# Autodesk Inventor assembly: Vex Traction Wheel 4x2
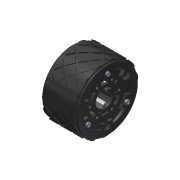
[picture p0: Inventor's stored thumbnail of the model, 180x180]
Saved by Autodesk Inventor 2013 (Build 170138000, 138)
## iProperties
Created: 2012-12-09
Part Number: Vex Traction Wheel 4x2
Document SubType Name: Assembly
Designer: Nemo
Author: Nemo
## Documents named in this file (7)
- H:\Nemo\Documents\Robotics\VexPro\Wheels\Assemblies\Vex Traction Wheel 4x2.iam
- H:\Nemo\Documents\Robotics\VexPro\Wheels\Components\Traction Tire Body 4in.ipt
- H:\Nemo\Documents\Robotics\VexPro\Wheels\Components\Traction Tire extension 4in.ipt
- H:\Nemo\Documents\Robotics\VexPro\Fasteners\8-32 locknut.ipt
- H:\Nemo\Documents\Robotics\VexPro\Fasteners\Hex Standoff 8-32 x1750.ipt
- H:\Nemo\Documents\Robotics\VexPro\Fasteners\8-32 SHCS x2250.ipt
- H:\Nemo\Documents\Robotics\VexPro\Wheels\Components\4 Traction Tire - 2 Wide.ipt
## Components (17 placed, 6 different names)
1. Traction Tire Body 4in:1 — Mate:1, Mate:2, Mate:3, Mate:4, Mate:5, Mate:6, Mate:9, Angle:1, Mate:10, Insert:2, Angle:2
2. Traction Tire Body 4in:2 — Mate:3, Mate:7, Insert:1, Mate:12, Insert:4
3. Traction Tire extension 4in:1 — Mate:4, Mate:5, Mate:6, Mate:7, Flush:1, Insert:3
4. Traction Tire extension 4in:2 — Mate:11, Insert:3, Mate:12
5. 4 Traction Tire - 2 Wide:1 — Mate:13, Mate:14, Mate:15
6. Hex Standoff 8-32 x1750:1 — Mate:9, Angle:1, Mate:10
7. Hex Standoff 8-32 x1750:2
8. Hex Standoff 8-32 x1750:3
9. Hex Standoff 8-32 x1750:4
10. Hex Standoff 8-32 x1750:5
11. Hex Standoff 8-32 x1750:6
12. 8-32 SHCS x2250:1 — Insert:1, Insert:4
13. 8-32 locknut:1 — Insert:2, Angle:2
14. 8-32 SHCS x2250:2
15. 8-32 locknut:2
16. 8-32 SHCS x2250:3
17. 8-32 locknut:3
## Component patterns: (6 elements, first: Hex Standoff 8-32 x1750:1), (3 elements, first: 8-32 SHCS x2250:1 + 8-32 locknut:1)
## Relationships (21: Mate 14, Insert 4, Angle 2, Flush 1)
- Mate:1: Traction Tire Body 4in:1
- Mate:2: Traction Tire Body 4in:1
- Mate:3: Traction Tire Body 4in:1 ↔ Traction Tire Body 4in:2
- Mate:4: Traction Tire Body 4in:1 ↔ Traction Tire extension 4in:1
- Mate:5: Traction Tire Body 4in:1 ↔ Traction Tire extension 4in:1
- Mate:6: Traction Tire Body 4in:1 ↔ Traction Tire extension 4in:1
- Mate:7: Traction Tire Body 4in:2 ↔ Traction Tire extension 4in:1
- Mate:9: Traction Tire Body 4in:1 ↔ Hex Standoff 8-32 x1750:1
- Angle:1 (0 deg): Traction Tire Body 4in:1 ↔ Hex Standoff 8-32 x1750:1
- Mate:10: Traction Tire Body 4in:1 ↔ Hex Standoff 8-32 x1750:1
- Insert:1: Traction Tire Body 4in:2 ↔ 8-32 SHCS x2250:1
- Insert:2: Traction Tire Body 4in:1 ↔ 8-32 locknut:1
- Angle:2 (0 deg): Traction Tire Body 4in:1 ↔ 8-32 locknut:1
- Flush:1: Traction Tire extension 4in:1
- Mate:11: Traction Tire extension 4in:2
- Insert:3: Traction Tire extension 4in:1 ↔ Traction Tire extension 4in:2
- Mate:12: Traction Tire Body 4in:2 ↔ Traction Tire extension 4in:2
- Mate:13: 4 Traction Tire - 2 Wide:1
- Mate:14: 4 Traction Tire - 2 Wide:1
- Mate:15: 4 Traction Tire - 2 Wide:1
- Insert:4: Traction Tire Body 4in:2 ↔ 8-32 SHCS x2250:1
